# Autodesk Inventor assembly: KOSZYK
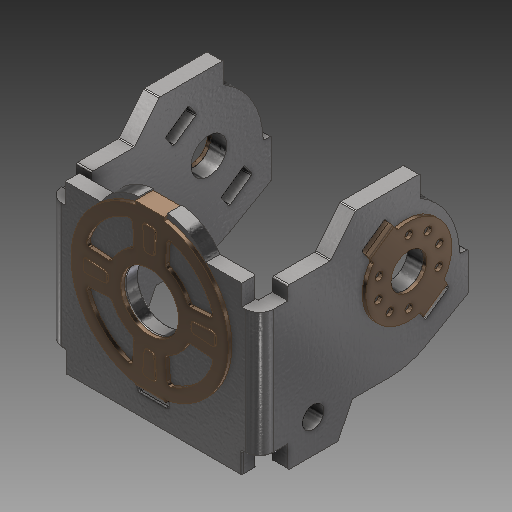
[picture p0: Inventor's stored thumbnail of the model, 512x512]
Saved by Autodesk Inventor 2017 SP1 (Build 210196100, 196)
## iProperties
Created: 2021-01-31
Part Number: KOSZYK
Document SubType Name: Assembly
Designer: Napoleon
Author: Napoleon
## Documents named in this file (4)
- D:\PRYWATNE\PROJEKTY\POKÓJ\URZĄDZENIA PERYFERYJNE\DELL 1909Wf\KOSZYK.iam
- D:\PRYWATNE\PROJEKTY\POKÓJ\URZĄDZENIA PERYFERYJNE\DELL 1909Wf\KOSZYK.ipt
- D:\PRYWATNE\PROJEKTY\POKÓJ\URZĄDZENIA PERYFERYJNE\DELL 1909Wf\SŁONECZKO KOSZYKA.ipt
- D:\PRYWATNE\PROJEKTY\POKÓJ\URZĄDZENIA PERYFERYJNE\DELL 1909Wf\SŁONECZKO MAŁE.ipt
## Components (4 placed, 3 different names)
1. KOSZYK:1 — Sztywne:2, Sztywne:3
2. SŁONECZKO KOSZYKA:1
3. SŁONECZKO MAŁE:1 — Sztywne:2
4. SŁONECZKO MAŁE:2 — Sztywne:3
## Relationships (2: WeldJoint 2)
- Sztywne:2 [WeldJoint]: KOSZYK:1 ↔ SŁONECZKO MAŁE:1
- Sztywne:3 [WeldJoint]: KOSZYK:1 ↔ SŁONECZKO MAŁE:2
